# Autodesk Inventor assembly: ELMA+K60-S210+K60-S150
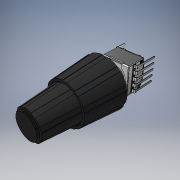
[picture p0: Inventor's stored thumbnail of the model, 180x180]
Saved by Autodesk Inventor 2018 (Build 220112000, 112)
## iProperties
Created: 2020-04-24
Part Number: ELMA+K60-S210+K60-S150
Material: Všeobecné
Document SubType Name: Assembly
Designer: Jozko Mrkvicka
Author: Jozko Mrkvicka
## Documents named in this file (4)
- F:\Workspace\Projekty\Library\ELMA+K60-S210+K60-S150.iam
- F:\Workspace\Projekty\Library\ELMA-E37.ipt
- F:\Workspace\Projekty\Library\Knob-K60-S150.ipt
- F:\Workspace\Projekty\Library\Knob-K60-S210.ipt
## Components (3 placed, 3 different names)
1. ELMA-E37:1 — Vložit:3, Proti sobě:1, Proti sobě:2
2. Knob-K60-S150:1 — Proti sobě:1, Proti sobě:2
3. Knob-K60-S210:1 — Vložit:3
## Relationships (3: Mate 2, Insert 1)
- Vložit:3 [Insert]: ELMA-E37:1 ↔ Knob-K60-S210:1
- Proti sobě:1 [Mate]: ELMA-E37:1 ↔ Knob-K60-S150:1
- Proti sobě:2 [Mate] (0.2 mm): ELMA-E37:1 ↔ Knob-K60-S150:1
